# Autodesk Inventor assembly: Left Idler Assembly
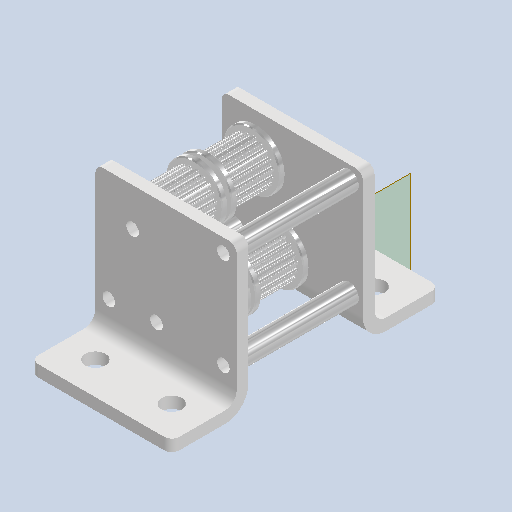
[picture p0: Inventor's stored thumbnail of the model, 512x512]
Saved by Autodesk Inventor 2024 (Build 280153000, 153)
## iProperties
Created: 2024-12-28
Part Number: Left Idler Assembly
Document SubType Name: Assembly
Designer: Ishaan
Author: Ishaan
## Documents named in this file (6)
- E:\Projects\Axiom--IDEX-3D-Printer\CAD\04 - Gantry\Left Idler Assembly.iam
- E:\Projects\Axiom--IDEX-3D-Printer\CAD\04 - Gantry\XY Idler Mount A.ipt
- E:\Projects\Axiom--IDEX-3D-Printer\CAD\00 - COTS Components\Hardware\M3 30mm Standoff.ipt
- E:\Projects\Axiom--IDEX-3D-Printer\CAD\00 - COTS Components\Hardware\M5 Shim 0p5mm.ipt
- E:\Projects\Axiom--IDEX-3D-Printer\CAD\00 - COTS Components\10mm 20T GT2 Idler Pulley 5mm Bore\10mm 20T GT2 Idler Pulley 5mm Bore.ipt
- E:\Projects\Axiom--IDEX-3D-Printer\CAD\04 - Gantry\XY Idler Mount B.ipt
## Components (17 placed, 5 different names)
1. XY Idler Mount A:1 — Insert:1, Insert:2, Insert:3, Insert:4, Insert:5, Insert:6, Insert:7
2. M3 30mm Standoff:1 — Insert:5
3. M3 30mm Standoff:2 — Insert:4
4. M3 30mm Standoff:3 — Insert:3, Insert:13
5. M3 30mm Standoff:4 — Insert:2, Insert:12
6. M3 30mm Standoff:5 — Insert:1
7. M5 Shim 0p5mm:1 — Insert:15, Insert:17
8. M5 Shim 0p5mm:2 — Insert:14, Insert:16
9. M5 Shim 0p5mm:3 — Insert:11
10. M5 Shim 0p5mm:4 — Insert:10
11. M5 Shim 0p5mm:5 — Insert:7, Insert:9
12. M5 Shim 0p5mm:6 — Insert:6, Insert:8
13. 10mm 20T GT2 Idler Pulley 5mm Bore:1 — Insert:8, Insert:11
14. 10mm 20T GT2 Idler Pulley 5mm Bore:2 — Insert:9, Insert:10
15. 10mm 20T GT2 Idler Pulley 5mm Bore:3 — Insert:17
16. 10mm 20T GT2 Idler Pulley 5mm Bore:4 — Insert:16
17. XY Idler Mount B:1 — Insert:12, Insert:13, Insert:14, Insert:15
## Relationships (17: Insert 17)
- Insert:1: XY Idler Mount A:1 ↔ M3 30mm Standoff:5
- Insert:2: XY Idler Mount A:1 ↔ M3 30mm Standoff:4
- Insert:3: XY Idler Mount A:1 ↔ M3 30mm Standoff:3
- Insert:4: XY Idler Mount A:1 ↔ M3 30mm Standoff:2
- Insert:5: XY Idler Mount A:1 ↔ M3 30mm Standoff:1
- Insert:6: XY Idler Mount A:1 ↔ M5 Shim 0p5mm:6
- Insert:7: XY Idler Mount A:1 ↔ M5 Shim 0p5mm:5
- Insert:8: M5 Shim 0p5mm:6 ↔ 10mm 20T GT2 Idler Pulley 5mm Bore:1
- Insert:9: M5 Shim 0p5mm:5 ↔ 10mm 20T GT2 Idler Pulley 5mm Bore:2
- Insert:10: M5 Shim 0p5mm:4 ↔ 10mm 20T GT2 Idler Pulley 5mm Bore:2
- Insert:11: M5 Shim 0p5mm:3 ↔ 10mm 20T GT2 Idler Pulley 5mm Bore:1
- Insert:12: M3 30mm Standoff:4 ↔ XY Idler Mount B:1
- Insert:13: M3 30mm Standoff:3 ↔ XY Idler Mount B:1
- Insert:14: M5 Shim 0p5mm:2 ↔ XY Idler Mount B:1
- Insert:15: M5 Shim 0p5mm:1 ↔ XY Idler Mount B:1
- Insert:16: M5 Shim 0p5mm:2 ↔ 10mm 20T GT2 Idler Pulley 5mm Bore:4
- Insert:17: M5 Shim 0p5mm:1 ↔ 10mm 20T GT2 Idler Pulley 5mm Bore:3
